# Autodesk Inventor assembly: Foot-40x
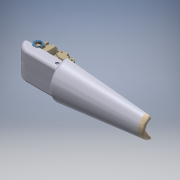
[picture p0: Inventor's stored thumbnail of the model, 180x180]
Saved by Autodesk Inventor 2018 (Build 220112000, 112)
## iProperties
Created: 2017-08-24
Part Number: Foot-40x
Material: Generisch
Document SubType Name: Assembly
Designer: JochenAlt
Author: JochenAlt
## Documents named in this file (4)
- D:\Projects\Manfred\design\cad\Inventor\Foot-40x.iam
- D:\Projects\Manfred\design\cad\Inventor\Foot-40x.ipt
- D:\Projects\Manfred\design\cad\Inventor\Rillenkugellager 11x7x3 inafag smr117.ipt
- D:\Projects\Manfred\design\cad\Inventor\Herkulex DRS-010x\HerkuleX DRS-0101.iam
## Components (3 placed, 3 different names)
1. Rillenkugellager 11x7x3 inafag smr117:1 — Passend:7, Passend:10
2. HerkuleX DRS-0101:1 [sub-assembly] — Passend:6, Winkel:1, Passend:9, Passend:10
3. Foot-40x:1 — Passend:6, Passend:7, Winkel:1, Passend:9
## Relationships (5: Mate 4, Angle 1)
- Passend:6 [Mate]: HerkuleX DRS-0101:1 ↔ Foot-40x:1
- Passend:7 [Mate]: Rillenkugellager 11x7x3 inafag smr117:1 ↔ Foot-40x:1
- Winkel:1 [Angle] (0 deg): HerkuleX DRS-0101:1 ↔ Foot-40x:1
- Passend:9 [Mate] (0.1 mm): HerkuleX DRS-0101:1 ↔ Foot-40x:1
- Passend:10 [Mate] (0.1 mm): Rillenkugellager 11x7x3 inafag smr117:1 ↔ HerkuleX DRS-0101:1
